# Autodesk Inventor assembly: 1470706 EPCO-25-300-3P-ST-E---(0)
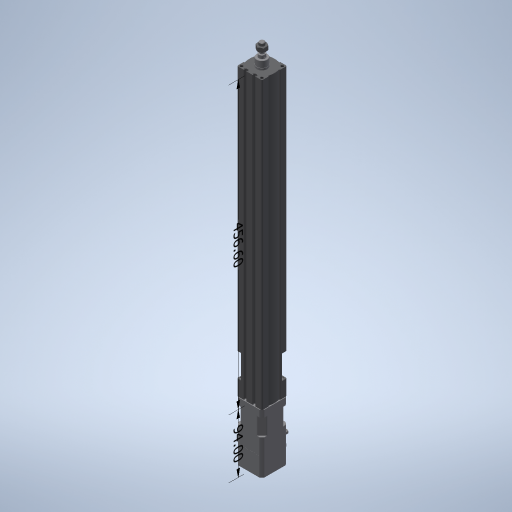
[picture p0: Inventor's stored thumbnail of the model, 512x512]
Saved by Autodesk Inventor 2023 (Build 270158000, 158)
## iProperties
Created: 2023-04-07
Part Number: 1470706 EPCO-25-300-3P-ST-E---(0)
Catalog Web Link: www.cadenas.de
Description: EPCO-electric cylinder
Vendor: FESTO
Document SubType Name: Assembly
Designer: psAdmin
Manufacturer: FESTO
Mass: 2524 g
Surface Area: 1754.44 cm^2
Volume: 669.022 cm^3
Density: 3.77267 g/cm^3
Category: PARTsolutions
Company: FESTO
PSOL_IDENT_0: {$CADENAS_DATA/23d-libs/festo/parts/e/epco/epco_asmtab_presets.prj},223 {VTYP=3D},{STYP=ASSTAB},{NB=
PSOL_IDENT_1: 1470706 EPCO-25-300-3P-ST-E---(0)},{LINA=1470706 EPCO-25-300-3P-ST-E},{NN=EPCO},{DATE=22.03.2023 08:
PSOL_IDENT_2: 58:34},{GEOMDATE=16.03.2023 11:33:05},{VERSION=},{LINEID=160},{WBVAR=HUBST},{WBNUMERIC=HUBST}  {NB=1
PSOL_IDENT_3: 470706 EPCO-25-300-3P-ST-E---(0)},{LINA=1470706 EPCO-25-300-3P-ST-E},{KT=DUMMY},{TNR=1470706},{TYP=E
PSOL_IDENT_4: PCO-25},{INFO=2025-12-31},{KDM=25},{HUB=300},{HUBST=0},{SPI=3P},{KOL=1},{KOLT=},{KOLB=0},{KOLB1=0},{
PSOL_IDENT_5: KOLBT=},{POS=-},{POST=},{MOT=ST},{MES=2},{MEST=-E},{BRE=1},{BRET=},{OA=0},{OAT=},{BED=-},{BEDT=},{MT
PSOL_IDENT_6: RTNR=1460675},{DIN934D=8.000},{DIN934P=1.000},{DIN912D=3.000},{DIN912L=25.000},{PPATH=assemblies/epc
PSOL_IDENT_7: o_asmtpl.prj},{AM=16},{B1=40},{B2=32.500},{D1=17.270},{D2=10},{D3=M5},{H1=42.000},{H2=40},{H3=32.500
PSOL_IDENT_8: },{KK=M8},{L1=474.6},{L11=174.600},{L2=456.6},{L22=156.600},{L3=94.4},{L4=18.000},{L5=4.200},{L6=12}
PSOL_IDENT_9: ,{SW1=9},{SW2=13},{CNSMASSEXACT=2.524},{GEWG=2.223},{GEWB=0.301},{GEW1=1.125},{GEW2=3.400},{GEW3=0.2
PSOL_IDENT_10: 60},{GEW11=0.145},{GEW22=0.260},{GEW33=0.260},{IDCODE=EPCO-25-300-3P-ST-E},{EOLDATE=31.12.2025}
NB: 1470706 EPCO-25-300-3P-ST-E---(0)
NN: EPCO
NT: electric cylinder
NBSYN: $TNR. $TYP.-$HUB.-$SPI.$KOLT.$KOLBT.$POST.-$MOT.$MEST.$BRET.$OAT.$BEDT.---($HUBST.)
LINA: 1470706 EPCO-25-300-3P-ST-E
CATALOG: Festo
TNR: 1470706
TYP: EPCO-25
INFO: 2025-12-31
HUB: 300
HUBST: 0
SPI: 3P
MOT: ST
AM: 16
B1: 40
B2: 32.5
D1: 17.27
D2: 10
D3: M5
H1: 42
H2: 40
H3: 32.5
KK: M8
L1: 474.6
L2: 456.6
L3: 94.4
L4: 18
L5: 4.2
L6: 12
SW1: 9
SW2: 13
CNSMASSEXACT: 2.524
SUPPLIER: FESTO
ARTICLENO: 1470706 EPCO-25-300-3P-ST-E---(0)
BOMINFO: 1470706 EPCO-25-300-3P-ST-E
CREATOR: CADENAS GmbH
Title: 1470706 EPCO-25-300-3P-ST-E
Author: Cadenas PARTsolutions
Comments: electric cylinder
## Documents named in this file (6)
- D:\Esdek\Gemelo Digital\Corte de Tubos\CADimportados\PistónElectromecánico\1470706 EPCO-25-300-3P-ST-E---(0).iam
- D:\Esdek\Gemelo Digital\Corte de Tubos\CADimportados\PistónElectromecánico\1470874 EPCO-25-30000_z---(0).ipt
- D:\Esdek\Gemelo Digital\Corte de Tubos\CADimportados\PistónElectromecánico\1470874 EPCO-25-300_k---(1_0).ipt
- D:\Esdek\Gemelo Digital\Corte de Tubos\CADimportados\PistónElectromecánico\DIN 934 - M8x1(F).ipt
- D:\Esdek\Gemelo Digital\Corte de Tubos\CADimportados\PistónElectromecánico\1460675 EMMS-ST-42-SS-SE-G2.ipt
- D:\Esdek\Gemelo Digital\Corte de Tubos\CADimportados\PistónElectromecánico\DIN-912 - M3x25(F).ipt
## Components (6 placed, 5 different names)
1. 1470874 EPCO-25-30000_z---(0):1 — TO_KS_XY@1 <-> EPCO_KS_XY@2, TO_KS_Z@1 <-> EPCO_KS_Z@2, TO_KS_YZ@1 <-> EPCO_KS_YZ@2, TO_MOTOR_XY@1 <-> ANBAU_XY@4, TO_MOTOR_Z@1 <-> ANBAU_Z@4, TO_MOTOR_YZ@1 <-> ANBAU_YZ@4, SCREW_1_XY@1 <-> ANBAU_XY@5, SCREW_1_Z@1 <-> ANBAU_Z@5, SCREW_1_YZ@1 <-> ANBAU_YZ@5, SCREW_2_XY@1 <-> ANBAU_XY@6, SCREW_2_Z@1 <-> ANBAU_Z@6, SCREW_2_YZ@1 <-> ANBAU_YZ@6
2. 1470874 EPCO-25-300_k---(1_0):1 — TO_KS_XY@1 <-> EPCO_KS_XY@2, TO_KS_Z@1 <-> EPCO_KS_Z@2, TO_KS_YZ@1 <-> EPCO_KS_YZ@2, NUT_XY@2 <-> IPunten_XY@3, NUT_Z@2 <-> IPunten_Z@3, NUT_YZ@2 <-> IPunten_YZ@3
3. DIN 934 - M8x1(F):1 — NUT_XY@2 <-> IPunten_XY@3, NUT_Z@2 <-> IPunten_Z@3, NUT_YZ@2 <-> IPunten_YZ@3
4. 1460675 EMMS-ST-42-SS-SE-G2:1 — TO_MOTOR_XY@1 <-> ANBAU_XY@4, TO_MOTOR_Z@1 <-> ANBAU_Z@4, TO_MOTOR_YZ@1 <-> ANBAU_YZ@4
5. DIN-912 - M3x25(F):1 — SCREW_1_XY@1 <-> ANBAU_XY@5, SCREW_1_Z@1 <-> ANBAU_Z@5, SCREW_1_YZ@1 <-> ANBAU_YZ@5
6. DIN-912 - M3x25(F):2 — SCREW_2_XY@1 <-> ANBAU_XY@6, SCREW_2_Z@1 <-> ANBAU_Z@6, SCREW_2_YZ@1 <-> ANBAU_YZ@6
## Relationships (15: Mate 10, Angle 5)
- TO_KS_XY@1 <-> EPCO_KS_XY@2 [Mate]: 1470874 EPCO-25-30000_z---(0):1 ↔ 1470874 EPCO-25-300_k---(1_0):1
- TO_KS_Z@1 <-> EPCO_KS_Z@2 [Mate]: 1470874 EPCO-25-30000_z---(0):1 ↔ 1470874 EPCO-25-300_k---(1_0):1
- TO_KS_YZ@1 <-> EPCO_KS_YZ@2 [Angle] (0 deg): 1470874 EPCO-25-30000_z---(0):1 ↔ 1470874 EPCO-25-300_k---(1_0):1
- NUT_XY@2 <-> IPunten_XY@3 [Mate] (3 mm): 1470874 EPCO-25-300_k---(1_0):1 ↔ DIN 934 - M8x1(F):1
- NUT_Z@2 <-> IPunten_Z@3 [Mate]: 1470874 EPCO-25-300_k---(1_0):1 ↔ DIN 934 - M8x1(F):1
- NUT_YZ@2 <-> IPunten_YZ@3 [Angle] (0 deg): 1470874 EPCO-25-300_k---(1_0):1 ↔ DIN 934 - M8x1(F):1
- TO_MOTOR_XY@1 <-> ANBAU_XY@4 [Mate]: 1470874 EPCO-25-30000_z---(0):1 ↔ 1460675 EMMS-ST-42-SS-SE-G2:1
- TO_MOTOR_Z@1 <-> ANBAU_Z@4 [Mate]: 1470874 EPCO-25-30000_z---(0):1 ↔ 1460675 EMMS-ST-42-SS-SE-G2:1
- TO_MOTOR_YZ@1 <-> ANBAU_YZ@4 [Angle] (0 deg): 1470874 EPCO-25-30000_z---(0):1 ↔ 1460675 EMMS-ST-42-SS-SE-G2:1
- SCREW_1_XY@1 <-> ANBAU_XY@5 [Mate]: 1470874 EPCO-25-30000_z---(0):1 ↔ DIN-912 - M3x25(F):1
- SCREW_1_Z@1 <-> ANBAU_Z@5 [Mate]: 1470874 EPCO-25-30000_z---(0):1 ↔ DIN-912 - M3x25(F):1
- SCREW_1_YZ@1 <-> ANBAU_YZ@5 [Angle] (0 deg): 1470874 EPCO-25-30000_z---(0):1 ↔ DIN-912 - M3x25(F):1
- SCREW_2_XY@1 <-> ANBAU_XY@6 [Mate]: 1470874 EPCO-25-30000_z---(0):1 ↔ DIN-912 - M3x25(F):2
- SCREW_2_Z@1 <-> ANBAU_Z@6 [Mate]: 1470874 EPCO-25-30000_z---(0):1 ↔ DIN-912 - M3x25(F):2
- SCREW_2_YZ@1 <-> ANBAU_YZ@6 [Angle] (0 deg): 1470874 EPCO-25-30000_z---(0):1 ↔ DIN-912 - M3x25(F):2
